# Autodesk Inventor assembly: table_assembly
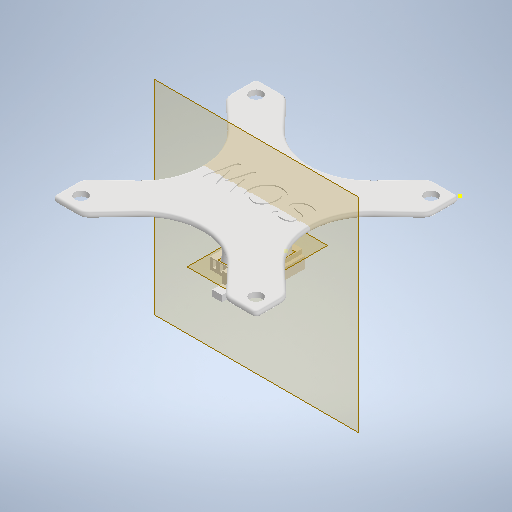
[picture p0: Inventor's stored thumbnail of the model, 512x512]
Saved by Autodesk Inventor 2025.2 (Build 292293000, 293)
## iProperties
Created: 2024-12-28
Part Number: table_assembly
Document SubType Name: Assembly
Designer: holz
Author: holz
## Documents named in this file (4)
- C:\Users\holz\Desktop\table_moving\table_assembly.iam
- C:\Users\holz\Desktop\table_moving\table_bridge.ipt
- C:\Users\holz\Desktop\table_moving\table_column.ipt
- C:\Users\holz\Desktop\table_moving\table_top.ipt
## Components (6 placed, 3 different names)
1. table_column:1 — Mate:5
2. table_column:2 — Mate:3
3. table_column:3 — Mate:4
4. table_column:4 — Mate:2
5. table_top:1
6. table_bridge:2
## Relationships (4: Mate 4)
- Mate:2: table_column:4
- Mate:3: table_column:2
- Mate:4: table_column:3
- Mate:5: table_column:1
